# Autodesk Inventor assembly: Montagem
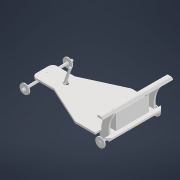
[picture p0: Inventor's stored thumbnail of the model, 180x180]
Saved by Autodesk Inventor 2022 (Build 260153000, 153)
## iProperties
Created: 2022-06-09
Part Number: Montagem
Document SubType Name: Assembly
Designer: Gugarauj07
Author: Gugarauj07
## Documents named in this file (10)
- C:\Users\Gugarauj07\PycharmProjects\Eletronica_2022\CADS\Carrinho_Rolima\Montagem\Montagem.iam
- C:\Users\Gugarauj07\PycharmProjects\Eletronica_2022\CADS\Carrinho_Rolima\Base.ipt
- C:\Users\Gugarauj07\PycharmProjects\Eletronica_2022\CADS\Carrinho_Rolima\Eixo_dianteiro.ipt
- C:\Users\Gugarauj07\PycharmProjects\Eletronica_2022\CADS\Carrinho_Rolima\Eixo_traseiro.ipt
- C:\Users\Gugarauj07\PycharmProjects\Eletronica_2022\CADS\Carrinho_Rolima\Base_Aerofoil.ipt
- C:\Users\Gugarauj07\PycharmProjects\Eletronica_2022\CADS\Carrinho_Rolima\Topo_Aerofoil.ipt
- C:\Users\Gugarauj07\PycharmProjects\Eletronica_2022\CADS\Carrinho_Rolima\Fixacao_FreioDianteiro.ipt
- C:\Users\Gugarauj07\PycharmProjects\Eletronica_2022\CADS\Carrinho_Rolima\Banco.ipt
- C:\Users\Gugarauj07\PycharmProjects\Eletronica_2022\CADS\Carrinho_Rolima\freio rolimã, como tu e tua irmã.ipt
- C:\Users\Gugarauj07\PycharmProjects\Eletronica_2022\CADS\Carrinho_Rolima\Roda.ipt
## Components (14 placed, 9 different names)
1. Base:1 — Mate:1, Mate:2, Mate:3, Mate:4, Mate:5, Mate:8, Mate:9, Mate:10
2. Eixo_dianteiro:1 — Mate:1, Mate:12, Mate:13
3. Eixo_traseiro:1 — Mate:2, Mate:3, Mate:14, Mate:15
4. Base_Aerofoil:1 — Mate:4, Mate:6, Mate:7
5. Base_Aerofoil:2 — Mate:5
6. Topo_Aerofoil:1 — Mate:6, Mate:7
7. Fixacao_FreioDianteiro:1 — Mate:8, Mate:11
8. Fixacao_FreioDianteiro:2 — Mate:9
9. Banco:1 — Mate:10
10. freio rolimã, como tu e tua irmã:1 — Mate:11
11. Roda:1 — Mate:12
12. Roda:2 — Mate:13
13. Roda:3 — Mate:14
14. Roda:4 — Mate:15
## Relationships (15: Mate 15)
- Mate:1: Base:1 ↔ Eixo_dianteiro:1
- Mate:2: Base:1 ↔ Eixo_traseiro:1
- Mate:3: Base:1 ↔ Eixo_traseiro:1
- Mate:4: Base:1 ↔ Base_Aerofoil:1
- Mate:5: Base:1 ↔ Base_Aerofoil:2
- Mate:6: Base_Aerofoil:1 ↔ Topo_Aerofoil:1
- Mate:7: Base_Aerofoil:1 ↔ Topo_Aerofoil:1
- Mate:8: Base:1 ↔ Fixacao_FreioDianteiro:1
- Mate:9: Base:1 ↔ Fixacao_FreioDianteiro:2
- Mate:10: Base:1 ↔ Banco:1
- Mate:11: Fixacao_FreioDianteiro:1 ↔ freio rolimã, como tu e tua irmã:1
- Mate:12: Eixo_dianteiro:1 ↔ Roda:1
- Mate:13: Eixo_dianteiro:1 ↔ Roda:2
- Mate:14: Eixo_traseiro:1 ↔ Roda:3
- Mate:15: Eixo_traseiro:1 ↔ Roda:4
